# Autodesk Inventor assembly: lensInHolder
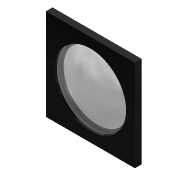
[picture p0: Inventor's stored thumbnail of the model, 180x180]
Saved by Autodesk Inventor 2018 (Build 220112000, 112)
## iProperties
Created: 2017-03-28
Part Number: lensInHolder
Document SubType Name: Assembly
Designer: sawaiz
Author: sawaiz
## Documents named in this file (3)
- C:\Users\sawaiz\OneDrive\projects\modularRICH\lensInHolder.iam
- C:\Users\sawaiz\OneDrive\projects\modularRICH\sphericalLensHolder.ipt
- C:\Users\sawaiz\OneDrive\projects\modularRICH\EO-27-501-100mmDIAx200F-PCXCondenser.ipt
## Components (2 placed, 2 different names)
1. sphericalLensHolder:1 — Mate:1, Mate:2
2. EO-27-501-100mmDIAx200F-PCXCondenser:1 — Mate:1, Mate:2
## Relationships (2: Mate 2)
- Mate:1: sphericalLensHolder:1 ↔ EO-27-501-100mmDIAx200F-PCXCondenser:1
- Mate:2: sphericalLensHolder:1 ↔ EO-27-501-100mmDIAx200F-PCXCondenser:1
